# Autodesk Inventor assembly: Odometer_Assembly
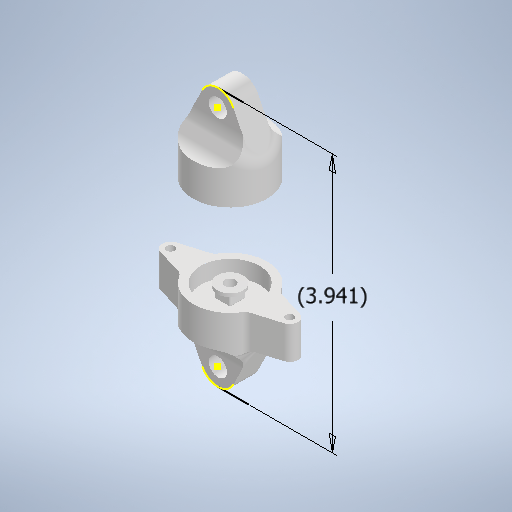
[picture p0: Inventor's stored thumbnail of the model, 512x512]
Saved by Autodesk Inventor 2025.1 (Build 291241020, 241B)
## iProperties
Created: 2024-10-31
Part Number: Odometer_Assembly
Document SubType Name: Assembly
Designer: AtuStem
Author: AtuStem
## Documents named in this file (4)
- C:\Users\AtuStem\Documents\GitHub\ATUM-V5RC-High-Stakes-CAD\Protobot\Odometer_Assembly.iam
- C:\Users\AtuStem\Documents\GitHub\ATUM-V5RC-High-Stakes-CAD\Protobot\Odom_Part1.ipt
- C:\Users\AtuStem\Documents\GitHub\ATUM-V5RC-High-Stakes-CAD\Protobot\Odom_Part1_Encoder.ipt
- C:\Users\AtuStem\Documents\GitHub\ATUM-V5RC-High-Stakes-CAD\VEX-CAD-Inventor\Motion\Insert Circle.ipt
## Components (4 placed, 3 different names)
1. Odom_Part1:1 — Mate:1, Flush:1
2. Odom_Part1_Encoder:1 — Mate:2, Flush:2
3. Insert Circle:1 — Mate:1, Flush:1, Mate:3
4. Insert Circle:2 — Mate:2, Flush:2, Mate:3
## Relationships (5: Mate 3, Flush 2)
- Mate:1: Odom_Part1:1 ↔ Insert Circle:1
- Flush:1: Odom_Part1:1 ↔ Insert Circle:1
- Mate:2: Odom_Part1_Encoder:1 ↔ Insert Circle:2
- Flush:2: Odom_Part1_Encoder:1 ↔ Insert Circle:2
- Mate:3: Insert Circle:1 ↔ Insert Circle:2
